# Autodesk Inventor assembly: dummy_zestaw
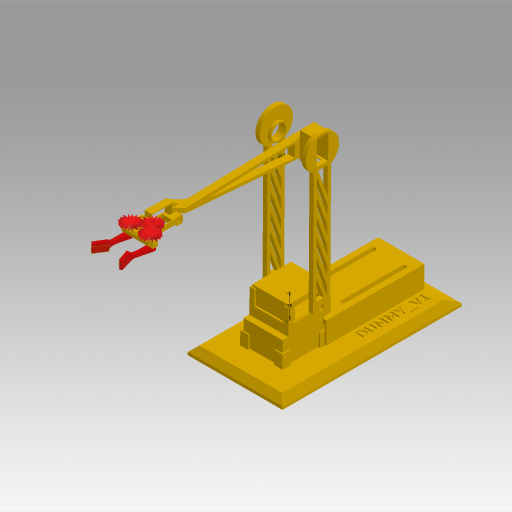
[picture p0: Inventor's stored thumbnail of the model, 512x512]
Saved by Autodesk Inventor 2024.3 (Build 283343000, 343)
## iProperties
Created: 2024-07-28
Part Number: dummy_zestaw
Document SubType Name: Assembly
Designer: User
Author: User
## Documents named in this file (13)
- C:\Users\Duszy\Desktop\Dummy_v1\dummy_zestaw.iam
- C:\Users\Duszy\Desktop\Dummy_v1\baza.ipt
- C:\Users\Duszy\Desktop\Dummy_v1\Część4.ipt
- C:\Users\Duszy\Desktop\Dummy_v1\Część5.ipt
- C:\Users\Duszy\Desktop\Dummy_v1\Część6.ipt
- C:\Users\Duszy\Desktop\Dummy_v1\arm_v3-1_backup.ipt
- C:\Users\Duszy\Desktop\Dummy_v1\arm_v3_backup.ipt
- C:\Users\Duszy\Desktop\Dummy_v1\pointrer.ipt
- C:\Users\Duszy\Desktop\Dummy_v1\proto_szczypce.ipt
- C:\Users\Duszy\Desktop\Dummy_v1\GEAR.ipt
- C:\Users\Duszy\Desktop\Dummy_v1\GEAR_SERV.ipt
- C:\Users\Duszy\Desktop\Dummy_v1\klapa.ipt
- C:\Users\Duszy\Desktop\Dummy_v1\huj.ipt
## Components (14 placed, 12 different names)
1. baza:1 — przesuwne:1, Sztywne:2
2. Część4:1 — Sztywne:1, Obrotowe:2, Obrotowe:3
3. Część5:1 — Obrotowe:1, Sztywne:1
4. Część6:1 — Obrotowe:1, przesuwne:1
5. arm_v3-1_backup:1 — Obrotowe:2, Obrotowe:5, Obrotowe:7
6. arm_v3_backup:1 — Obrotowe:3, Obrotowe:4
7. pointrer:1 — Obrotowe:4, Obrotowe:5, Obrotowe:6, Obrotowe:7, Obrotowe:8
8. proto_szczypce:1 — Obrotowe:6, Obrotowe:8, Obrotowe:9, Obrotowe:10, Obrotowe:11, Obrotowe:12, Obrotowe:13
9. GEAR_SERV:1 — Obrotowe:9, Obrót:1, Obrót:2
10. GEAR:1 — Obrotowe:10, Obrót:1
11. GEAR:2 — Obrotowe:11, Obrót:2
12. klapa:1 — Sztywne:2
13. huj:1 — Obrotowe:13
14. huj:2 — Obrotowe:12
## Relationships (18: RevoluteJoint 13, WeldJoint 2, RelateRotation 2, TranslationJoint 1)
- Obrotowe:1 [RevoluteJoint]: Część5:1 ↔ Część6:1
- Sztywne:1 [WeldJoint] (20 mm): Część4:1 ↔ Część5:1
- przesuwne:1 [TranslationJoint] (5 mm): baza:1 ↔ Część6:1
- Obrotowe:2 [RevoluteJoint] (-45 mm): Część4:1 ↔ arm_v3-1_backup:1
- Obrotowe:3 [RevoluteJoint] (-2 mm): Część4:1 ↔ arm_v3_backup:1
- Obrotowe:4 [RevoluteJoint] (-20 mm): arm_v3_backup:1 ↔ pointrer:1
- Obrotowe:5 [RevoluteJoint] (17 mm): arm_v3-1_backup:1 ↔ pointrer:1
- Obrotowe:6 [RevoluteJoint]: pointrer:1 ↔ proto_szczypce:1
- Obrotowe:7 [RevoluteJoint] (-22 mm): arm_v3-1_backup:1 ↔ pointrer:1
- Obrotowe:8 [RevoluteJoint]: pointrer:1 ↔ proto_szczypce:1
- Obrotowe:9 [RevoluteJoint]: proto_szczypce:1 ↔ GEAR_SERV:1
- Obrotowe:10 [RevoluteJoint] (5 mm): proto_szczypce:1 ↔ GEAR:1
- Obrót:1 [RelateRotation] (1 ul): GEAR_SERV:1 ↔ GEAR:1
- Obrotowe:11 [RevoluteJoint] (5 mm): proto_szczypce:1 ↔ GEAR:2
- Obrót:2 [RelateRotation] (1 ul): GEAR_SERV:1 ↔ GEAR:2
- Sztywne:2 [WeldJoint]: baza:1 ↔ klapa:1
- Obrotowe:12 [RevoluteJoint]: proto_szczypce:1 ↔ huj:2
- Obrotowe:13 [RevoluteJoint]: proto_szczypce:1 ↔ huj:1
